# Autodesk Inventor assembly: Ensamble_Prueba2
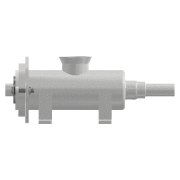
[picture p0: Inventor's stored thumbnail of the model, 180x180]
Saved by Autodesk Inventor 2021 (Build 250183000, 183)
## iProperties
Created: 2022-02-08
Part Number: Ensamble_Prueba2
Document SubType Name: Assembly
Designer: Santiago
Author: Santiago
## Documents named in this file (9)
- C:\Users\user\Desktop\Ingeniería Mecánica UN\7. Séptimo Semestre\Diseño de Elementos de Máquinas 1\Proyecto Moledora\Ensamble_Prueba2.iam
- C:\Users\user\Desktop\Ingeniería Mecánica UN\7. Séptimo Semestre\Diseño de Elementos de Máquinas 1\Proyecto Moledora\Tornillo Molienda.iam
- C:\Users\user\Desktop\Ingeniería Mecánica UN\7. Séptimo Semestre\Diseño de Elementos de Máquinas 1\Proyecto Moledora\Carcasa.ipt
- C:\Users\user\Desktop\Ingeniería Mecánica UN\7. Séptimo Semestre\Diseño de Elementos de Máquinas 1\Proyecto Moledora\PoleaX.ipt
- C:\Users\user\Desktop\Ingeniería Mecánica UN\7. Séptimo Semestre\Diseño de Elementos de Máquinas 1\Proyecto Moledora\Sujetador_Rodamiento.ipt
- C:\Users\user\Desktop\Ingeniería Mecánica UN\7. Séptimo Semestre\Diseño de Elementos de Máquinas 1\Proyecto Moledora\Ensamble_Prueba\Design Accelerator\Bearing1.iam
- C:\Users\user\Documents\Inventor\Content Center Files\R2021\en-US\ISO 7091\ISO 7091 - ST 6 - 100 HV.ipt
- C:\Users\user\Documents\Inventor\Content Center Files\R2021\en-US\ISO 4017(1)\ISO 4017 - M6 x 30 - ISO.ipt
- C:\Users\user\Documents\Inventor\Content Center Files\R2021\en-US\ISO 4035(2)\ISO 4035 - M6 - ISO.ipt
## Components (11 placed, 8 different names)
1. Tornillo Molienda:1 [sub-assembly] — Mate:2, Mate:3, Mate:4, Flush:1, Mate:5, Mate:7
2. Carcasa:1 — Mate:2, Mate:6, Mate:16, Mate:18, Mate:19, Mate:20, Mate:22, Mate:23
3. PoleaX:1 — Mate:3
4. Bearing:1 [sub-assembly] — Mate:4, Flush:1
5. Sujetador_Rodamiento:1 — Mate:5, Mate:6, Mate:7, Mate:17, Mate:21
6. ISO 4017 M6 x 30:1 — Insert:4
7. ISO 4017 M6 x 30:2 — Insert:3
8. ISO 7091 ST 6 - 100 HV:1 — Mate:20, Mate:21, Insert:4
9. ISO 4035 M6:1 — Mate:22, Mate:23
10. ISO 7091 ST 6 - 100 HV:2 — Mate:16, Mate:17, Insert:3
11. ISO 4035 M6:2 — Mate:18, Mate:19
## Relationships (17: Mate 14, Insert 2, Flush 1)
- Mate:2: Tornillo Molienda:1 ↔ Carcasa:1
- Mate:3: Tornillo Molienda:1 ↔ PoleaX:1
- Mate:4: Tornillo Molienda:1 ↔ Bearing:1
- Flush:1: Tornillo Molienda:1 ↔ Bearing:1
- Mate:5: Tornillo Molienda:1 ↔ Sujetador_Rodamiento:1
- Mate:6: Carcasa:1 ↔ Sujetador_Rodamiento:1
- Mate:7: Tornillo Molienda:1 ↔ Sujetador_Rodamiento:1
- Mate:16: Carcasa:1 ↔ ISO 7091 ST 6 - 100 HV:2
- Mate:17: Sujetador_Rodamiento:1 ↔ ISO 7091 ST 6 - 100 HV:2
- Insert:3: ISO 4017 M6 x 30:2 ↔ ISO 7091 ST 6 - 100 HV:2
- Mate:18: Carcasa:1 ↔ ISO 4035 M6:2
- Mate:19: Carcasa:1 ↔ ISO 4035 M6:2
- Mate:20: Carcasa:1 ↔ ISO 7091 ST 6 - 100 HV:1
- Mate:21: Sujetador_Rodamiento:1 ↔ ISO 7091 ST 6 - 100 HV:1
- Insert:4: ISO 4017 M6 x 30:1 ↔ ISO 7091 ST 6 - 100 HV:1
- Mate:22: Carcasa:1 ↔ ISO 4035 M6:1
- Mate:23: Carcasa:1 ↔ ISO 4035 M6:1
